# Autodesk Inventor assembly: Inner rails
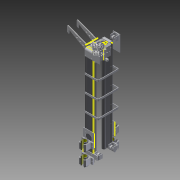
[picture p0: Inventor's stored thumbnail of the model, 180x180]
Saved by Autodesk Inventor 2013 (Build 170138000, 138)
## iProperties
Created: 2013-01-27
Part Number: Inner rails
Document SubType Name: Assembly
Designer: Arpan
Mass: 4602.07 g
Surface Area: 8094.53 cm^2
Volume: 1948.66 cm^3
Density: 2.36166 g/cm^3
Author: Arpan
## Documents named in this file (10)
- C:\Users\Arpan\Documents\GitHub\frc2013CAD\Cimber actual\Inner rails.iam
- C:\Users\Arpan\Documents\GitHub\frc2013CAD\Cimber actual\Shaft 26 inch.ipt
- C:\Users\Arpan\Documents\GitHub\frc2013CAD\Cimber actual\tie-together tier 1.ipt
- C:\Users\Arpan\Documents\GitHub\frc2013CAD\Cimber actual\upper face mount.ipt
- C:\Users\Arpan\Documents\GitHub\frc2013CAD\Cimber actual\face mount.ipt
- C:\Users\Arpan\Documents\GitHub\frc2013CAD\Cimber actual\bearing block short style.iam
- C:\Users\Arpan\Documents\GitHub\frc2013CAD\Cimber actual\hook block.iam
- C:\Users\Arpan\Documents\GitHub\frc2013CAD\Cimber actual\endstop 3.ipt
- C:\Users\Arpan\Documents\GitHub\frc2013CAD\Cimber actual\endstop 4.ipt
- C:\Users\Arpan\Documents\GitHub\frc2013CAD\Cimber actual\mini pulley assembly.iam
## Components (20 placed, 9 different names)
1. Shaft 26 inch:1 — Angle:1, Flush:1, Mate:15, Mate:22, Mate:23, Mate:31, Mate:32, Mate:47, Mate:48, Mate:49, Mate:50, Mate:58, Mate:61, Mate:62, Mate:63
2. Shaft 26 inch:2 — Angle:1, Flush:1, Mate:25, Mate:26, Mate:28, Mate:29, Mate:46, Flush:2, Mate:51, Mate:52, Mate:53, Mate:57, Mate:59, Mate:60
3. tie-together tier 1:2 — Mate:15, Mate:57
4. tie-together tier 1:3 — Mate:58, Mate:59, Mate:60
5. upper face mount:1 — Mate:25, Mate:26, Mate:42, Mate:43, Mate:44
6. upper face mount:2 — Mate:22, Mate:23, Mate:39, Mate:40, Mate:41
7. face mount:1 — Mate:28, Mate:29, Mate:36, Mate:37, Mate:38, Mate:64, Flush:7, Flush:8
8. face mount:2 — Mate:31, Mate:32, Mate:33, Mate:34, Mate:35, Mate:65, Flush:9, Flush:10
9. bearing block short style:1 [sub-assembly] — Mate:33, Mate:34, Mate:35
10. bearing block short style:2 [sub-assembly] — Mate:36, Mate:37, Mate:38
11. bearing block short style:3 [sub-assembly] — Mate:39, Mate:40, Mate:41
12. bearing block short style:4 [sub-assembly] — Mate:42, Mate:43, Mate:44
13. hook block:1 [sub-assembly] — Mate:46, Mate:47, Flush:2
14. endstop 3:1 — Mate:51, Mate:52, Mate:53, Mate:54, Flush:3, Flush:4
15. endstop 4:1 — Mate:48, Mate:49, Mate:50, Mate:55, Flush:5, Flush:6
16. mini pulley assembly:1 [sub-assembly] — Mate:54, Flush:3, Flush:4
17. mini pulley assembly:2 [sub-assembly] — Mate:55, Flush:5, Flush:6
18. tie-together tier 1:4 — Mate:61, Mate:62, Mate:63
19. mini pulley assembly:3 [sub-assembly] — Mate:64, Flush:7, Flush:8
20. mini pulley assembly:4 [sub-assembly] — Mate:65, Flush:9, Flush:10
## Relationships (51: Mate 40, Flush 10, Angle 1)
- Angle:1 (180 deg): Shaft 26 inch:1 ↔ Shaft 26 inch:2
- Flush:1: Shaft 26 inch:1 ↔ Shaft 26 inch:2
- Mate:15: Shaft 26 inch:1 ↔ tie-together tier 1:2
- Mate:22: Shaft 26 inch:1 ↔ upper face mount:2
- Mate:23: Shaft 26 inch:1 ↔ upper face mount:2
- Mate:25: Shaft 26 inch:2 ↔ upper face mount:1
- Mate:26: Shaft 26 inch:2 ↔ upper face mount:1
- Mate:28: Shaft 26 inch:2 ↔ face mount:1
- Mate:29: Shaft 26 inch:2 ↔ face mount:1
- Mate:31: Shaft 26 inch:1 ↔ face mount:2
- Mate:32: Shaft 26 inch:1 ↔ face mount:2
- Mate:33: face mount:2 ↔ bearing block short style:1
- Mate:34: face mount:2 ↔ bearing block short style:1
- Mate:35: face mount:2 ↔ bearing block short style:1
- Mate:36: face mount:1 ↔ bearing block short style:2
- Mate:37: face mount:1 ↔ bearing block short style:2
- Mate:38: face mount:1 ↔ bearing block short style:2
- Mate:39: upper face mount:2 ↔ bearing block short style:3
- Mate:40: upper face mount:2 ↔ bearing block short style:3
- Mate:41: upper face mount:2 ↔ bearing block short style:3
- Mate:42: upper face mount:1 ↔ bearing block short style:4
- Mate:43: upper face mount:1 ↔ bearing block short style:4
- Mate:44: upper face mount:1 ↔ bearing block short style:4
- Mate:46: Shaft 26 inch:2 ↔ hook block:1
- Mate:47: Shaft 26 inch:1 ↔ hook block:1
- Flush:2 (584.2 mm): Shaft 26 inch:2 ↔ hook block:1
- Mate:48: Shaft 26 inch:1 ↔ endstop 4:1
- Mate:49: Shaft 26 inch:1 ↔ endstop 4:1
- Mate:50: Shaft 26 inch:1 ↔ endstop 4:1
- Mate:51: Shaft 26 inch:2 ↔ endstop 3:1
- Mate:52: Shaft 26 inch:2 ↔ endstop 3:1
- Mate:53: Shaft 26 inch:2 ↔ endstop 3:1
- Mate:54: endstop 3:1 ↔ mini pulley assembly:1
- Flush:3: endstop 3:1 ↔ mini pulley assembly:1
- Flush:4: endstop 3:1 ↔ mini pulley assembly:1
- Mate:55: endstop 4:1 ↔ mini pulley assembly:2
- Flush:5: endstop 4:1 ↔ mini pulley assembly:2
- Flush:6: endstop 4:1 ↔ mini pulley assembly:2
- Mate:57: Shaft 26 inch:2 ↔ tie-together tier 1:2
- Mate:58: Shaft 26 inch:1 ↔ tie-together tier 1:3
- Mate:59: Shaft 26 inch:2 ↔ tie-together tier 1:3
- Mate:60: Shaft 26 inch:2 ↔ tie-together tier 1:3
- Mate:61: Shaft 26 inch:1 ↔ tie-together tier 1:4
- Mate:62: Shaft 26 inch:1 ↔ tie-together tier 1:4
- Mate:63: Shaft 26 inch:1 ↔ tie-together tier 1:4
- Mate:64: face mount:1 ↔ mini pulley assembly:3
- Flush:7: face mount:1 ↔ mini pulley assembly:3
- Flush:8: face mount:1 ↔ mini pulley assembly:3
- Mate:65: face mount:2 ↔ mini pulley assembly:4
- Flush:9: face mount:2 ↔ mini pulley assembly:4
- Flush:10: face mount:2 ↔ mini pulley assembly:4
